# Autodesk Inventor assembly: 202
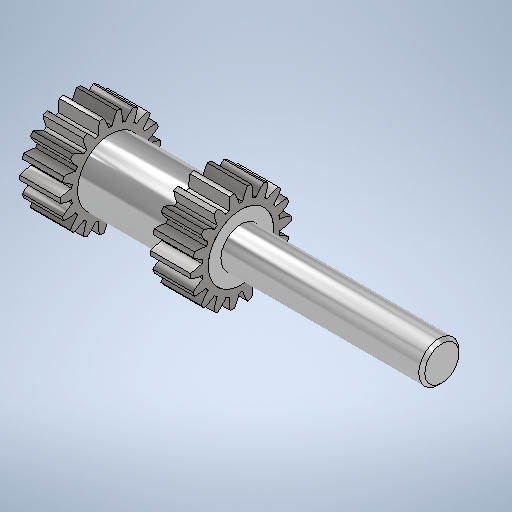
[picture p0: Inventor's stored thumbnail of the model, 512x512]
Saved by Autodesk Inventor 2025 (Build 290162010, 162A)
## iProperties
Created: 2024-07-12
Part Number: 202
Document SubType Name: Assembly
Designer: ffogue
Author: ffogue
## Documents named in this file (3)
- C:\Users\Fabri\Documents\Inventor\GearBox\202.iam
- C:\Users\Fabri\Documents\Inventor\GearBox\202 Welle.ipt
- C:\Users\Fabri\Documents\Inventor\GearBox\gear_204_18.iam
## Components (3 placed, 2 different names)
1. 202 Welle:1 — Insert:1, Insert:2
2. gear_204_18:1 [sub-assembly] — Insert:2
3. gear_204_18:2 [sub-assembly] — Insert:1
## Relationships (2: Insert 2)
- Insert:1 (-8 mm): 202 Welle:1 ↔ gear_204_18:2
- Insert:2 (-8 mm): 202 Welle:1 ↔ gear_204_18:1
